# Autodesk Inventor assembly: wings_MIR
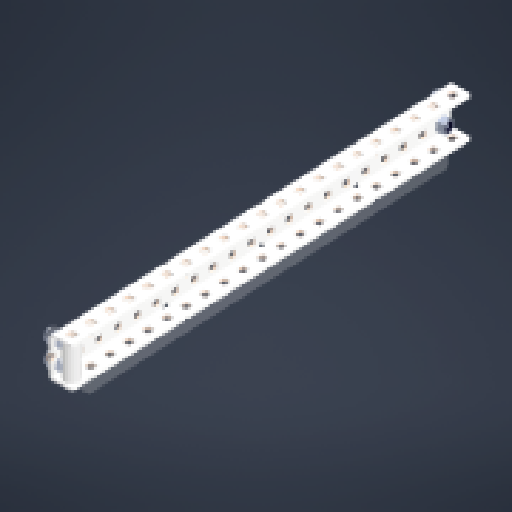
[picture p0: Inventor's stored thumbnail of the model, 512x512]
Saved by Autodesk Inventor 2023 (Build 270158000, 158)
## iProperties
Created: 2023-08-07
Part Number: wings_MIR
Document SubType Name: Assembly
Designer: srbel
Author: srbel
## Documents named in this file (9)
- C:\CAD\OverUnderCAD\Drive\wings_MIR.iam
- C:\CAD\OverUnderCAD\VEX-CAD-Inventor-1.4.0\Structure\C Channel\Aluminum 1x2x1\Alu C 1x2x1x21_MIR.ipt
- C:\CAD\OverUnderCAD\Drive\wingplexi_MIR.ipt
- C:\CAD\OverUnderCAD\VEX-CAD-Inventor-1.4.0\Structure\Hardware\Screw Steel - Star\SScrew Star Threaded .250.ipt
- C:\CAD\OverUnderCAD\VEX-CAD-Inventor-1.4.0\Structure\Hardware\Screw Steel - Star.ipt
- C:\CAD\OverUnderCAD\VEX-CAD-Inventor-1.4.0\Structure\Hardware\Nut Thin Nylock_MIR4.ipt
- C:\CAD\OverUnderCAD\VEX-CAD-Inventor-1.4.0\Motion\Spacers\Spacer Nylon .313 OD\NSpacer .313 OD x .500.ipt
- C:\CAD\OverUnderCAD\VEX-CAD-Inventor-1.4.0\Motion\Spacers\Spacer Nylon .313 OD.ipt
- C:\CAD\OverUnderCAD\VEX-CAD-Inventor-1.4.0\Motion\Spacers\Spacer Nylon .313 OD\NSpacer .313 OD x .375.ipt
## Components (12 placed, 6 different names)
1. Alu C 1x2x1x21_MIR:1 — Insert:2, Insert:1, Insert:9, Insert:10, Insert:11, Insert:12, Insert:13
2. wingplexi_MIR:1 — Insert:2, Insert:1, Insert:6, Insert:5, Insert:7, Insert:8
3. SScrew Star Threaded .250:1 — Insert:9
4. SScrew Star Threaded .250:2 — Insert:6
5. SScrew Star Threaded .250:3 — Insert:5
6. Nut Thin Nylock_MIR4:1 — Insert:7
7. Nut Thin Nylock_MIR4:2 — Insert:8
8. SScrew Star Threaded .250:4 — Insert:10
9. Nut Thin Nylock_MIR4:3 — Insert:11
10. Nut Thin Nylock_MIR4:4 — Insert:12
11. NSpacer .313 OD x .500:1 — Insert:14
12. NSpacer .313 OD x .375:2 — Insert:14, Insert:13
## Relationships (12: Insert 12)
- Insert:2: Alu C 1x2x1x21_MIR:1 ↔ wingplexi_MIR:1
- Insert:1: Alu C 1x2x1x21_MIR:1 ↔ wingplexi_MIR:1
- Insert:9: Alu C 1x2x1x21_MIR:1 ↔ SScrew Star Threaded .250:1
- Insert:6: wingplexi_MIR:1 ↔ SScrew Star Threaded .250:2
- Insert:5: wingplexi_MIR:1 ↔ SScrew Star Threaded .250:3
- Insert:7: wingplexi_MIR:1 ↔ Nut Thin Nylock_MIR4:1
- Insert:8: wingplexi_MIR:1 ↔ Nut Thin Nylock_MIR4:2
- Insert:10: Alu C 1x2x1x21_MIR:1 ↔ SScrew Star Threaded .250:4
- Insert:11: Alu C 1x2x1x21_MIR:1 ↔ Nut Thin Nylock_MIR4:3
- Insert:12: Alu C 1x2x1x21_MIR:1 ↔ Nut Thin Nylock_MIR4:4
- Insert:14: NSpacer .313 OD x .500:1 ↔ NSpacer .313 OD x .375:2
- Insert:13: Alu C 1x2x1x21_MIR:1 ↔ NSpacer .313 OD x .375:2
